# Autodesk Inventor assembly: BODY
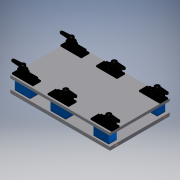
[picture p0: Inventor's stored thumbnail of the model, 180x180]
Saved by Autodesk Inventor 2017 (Build 210142000, 142)
## iProperties
Created: 2017-09-24
Part Number: BODY
Document SubType Name: Assembly
Designer: Alexander Miller
Author: Alexander Miller
## Documents named in this file (4)
- D:\Daten\Documents\Git\HeRo-Mini\Hardware\BODY.iam
- D:\Daten\Documents\Git\HeRo-Mini\Hardware\BODY_BOTTOM.ipt
- D:\Daten\Documents\Git\HeRo-Mini\Hardware\BODY_TOP.ipt
- D:\Daten\Documents\Git\HeRo-Mini\Hardware\SERVO.iam
## Components (8 placed, 3 different names)
1. BODY_BOTTOM:1 — Rigid:1, Rigid:2, Rigid:3, Rigid:4, Rigid:5, Rigid:6
2. BODY_TOP:1 — Rigid:7
3. SERVO:1 [sub-assembly] — Rigid:1, Rigid:7
4. SERVO:2 [sub-assembly] — Rigid:2
5. SERVO:3 [sub-assembly] — Rigid:3
6. SERVO:4 [sub-assembly] — Rigid:4
7. SERVO:5 [sub-assembly] — Rigid:5
8. SERVO:6 [sub-assembly] — Rigid:6
## Relationships (7: WeldJoint 7)
- Rigid:1 [WeldJoint]: BODY_BOTTOM:1 ↔ SERVO:1
- Rigid:2 [WeldJoint]: BODY_BOTTOM:1 ↔ SERVO:2
- Rigid:3 [WeldJoint]: BODY_BOTTOM:1 ↔ SERVO:3
- Rigid:4 [WeldJoint]: BODY_BOTTOM:1 ↔ SERVO:4
- Rigid:5 [WeldJoint]: BODY_BOTTOM:1 ↔ SERVO:5
- Rigid:6 [WeldJoint]: BODY_BOTTOM:1 ↔ SERVO:6
- Rigid:7 [WeldJoint]: BODY_TOP:1 ↔ SERVO:1
